# Autodesk Inventor assembly: Wheel And Motor
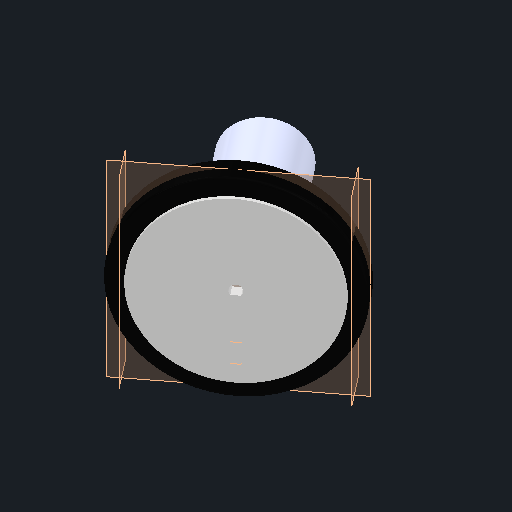
[picture p0: Inventor's stored thumbnail of the model, 512x512]
Saved by Autodesk Inventor 2026.2 (Build 302298000, 298)
## iProperties
Created: 2026-02-14
Part Number: Wheel And Motor
Document SubType Name: Assembly
Designer: chigg
Author: chigg
## Documents named in this file (4)
- C:\Users\chigg\Robot_Spring_Semester\Robot_Model\Wheel And Motor.iam
- C:\Users\chigg\Robot_Spring_Semester\Robot_Model\Swivel_Part.ipt
- C:\Users\chigg\Robot_Spring_Semester\Robot_Model\14)_Wheel.ipt
- C:\Users\chigg\Robot_Spring_Semester\Robot_Model\13)_Rubber Wheel Cap.ipt
## Components (3 placed, 3 different names)
1. Swivel_Part:1 — Insert:1
2. 14)_Wheel:1 — Mate:2, Mate:3, Insert:1, Flush:1
3. 13)_Rubber Wheel Cap:1 — Mate:2, Mate:3, Flush:1
## Relationships (4: Mate 2, Insert 1, Flush 1)
- Mate:2: 14)_Wheel:1 ↔ 13)_Rubber Wheel Cap:1
- Mate:3: 14)_Wheel:1 ↔ 13)_Rubber Wheel Cap:1
- Insert:1 (-10.0076 mm): Swivel_Part:1 ↔ 14)_Wheel:1
- Flush:1: 14)_Wheel:1 ↔ 13)_Rubber Wheel Cap:1
